# Autodesk Inventor assembly: X_CarriageR_V2_1
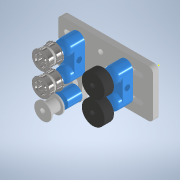
[picture p0: Inventor's stored thumbnail of the model, 180x180]
Saved by Autodesk Inventor 2021 (Build 250183000, 183)
## iProperties
Created: 2021-06-13
Part Number: X_CarriageR_V2_1
Document SubType Name: Assembly
Designer: Jorian Brusind
Author: Jorian Brusind
## Documents named in this file (9)
- C:\Users\Jorian Brusind\Documents\GitHub\PersonalProjects\HyperRail\Inventor Files\X_CarriageR_V2_1.iam
- C:\Users\Jorian Brusind\Documents\GitHub\PersonalProjects\HyperRail\Inventor Files\X_Carriage_Plate.ipt
- C:\Users\Jorian Brusind\Documents\GitHub\PersonalProjects\HyperRail\Inventor Files\Rollder_Spacer_Single.ipt
- C:\Users\Jorian Brusind\Documents\GitHub\PersonalProjects\HyperRail\Inventor Files\10mm_Idle_Pulley.ipt
- C:\Users\Jorian Brusind\Documents\GitHub\PersonalProjects\HyperRail\Inventor Files\4mm_Roller_Spacer_extended.ipt
- C:\Users\Jorian Brusind\Documents\GitHub\PersonalProjects\HyperRail\Inventor Files\11mm_BearingWheel.ipt
- C:\Users\Jorian Brusind\Documents\GitHub\PersonalProjects\HyperRail\Inventor Files\Bearing_Spacer.ipt
- C:\Users\Jorian Brusind\Documents\GitHub\PersonalProjects\HyperRail\Inventor Files\miniature-ball-bearings-metric-series-flanged-1.snapshot.1\F606ZZFlanged\F608 - 8 x 22 x 7.ipt
- C:\Users\Jorian Brusind\Documents\GitHub\PersonalProjects\HyperRail\Inventor Files\miniature-ball-bearings-metric-series-flanged-1.snapshot.1\F606ZZFlanged.ipt
## Components (13 placed, 7 different names)
1. X_Carriage_Plate:1 — Mate:35, Mate:67, Mate:69, Mate:72, Mate:84, Mate:85, Angle:1, Angle:2
2. Rollder_Spacer_Single:1 — Mate:35, Mate:40, Mate:42, Mate:67
3. 10mm_Idle_Pulley:1 — Mate:40, Mate:42
4. 4mm_Roller_Spacer_extended:1 — Mate:72, Mate:74, Mate:75, Mate:76, Mate:85, Angle:1
5. 4mm_Roller_Spacer_extended:3 — Mate:69, Mate:84, Angle:2, Mate:95, Mate:96, Mate:97
6. 11mm_BearingWheel:1 — Mate:75, Flush:1, Mate:76
7. 11mm_BearingWheel:2 — Mate:74, Flush:1
8. Bearing_Spacer:1 — Flush:3, Mate:92, Mate:93, Mate:94
9. Bearing_Spacer:2 — Flush:3, Mate:89, Mate:90, Mate:91
10. F608 - 8 x 22 x 7:1 — Mate:92, Mate:94, Mate:96
11. F608 - 8 x 22 x 7:2 — Mate:93
12. F608 - 8 x 22 x 7:3 — Mate:90
13. F608 - 8 x 22 x 7:4 — Mate:89, Mate:91, Mate:95, Mate:97
## Relationships (26: Mate 22, Flush 2, Angle 2)
- Mate:35: X_Carriage_Plate:1 ↔ Rollder_Spacer_Single:1
- Mate:40: Rollder_Spacer_Single:1 ↔ 10mm_Idle_Pulley:1
- Mate:42: Rollder_Spacer_Single:1 ↔ 10mm_Idle_Pulley:1
- Mate:67 (-18 mm): X_Carriage_Plate:1 ↔ Rollder_Spacer_Single:1
- Mate:69: X_Carriage_Plate:1 ↔ 4mm_Roller_Spacer_extended:3
- Mate:72: X_Carriage_Plate:1 ↔ 4mm_Roller_Spacer_extended:1
- Mate:74: 4mm_Roller_Spacer_extended:1 ↔ 11mm_BearingWheel:2
- Mate:75: 4mm_Roller_Spacer_extended:1 ↔ 11mm_BearingWheel:1
- Flush:1: 11mm_BearingWheel:1 ↔ 11mm_BearingWheel:2
- Mate:76: 4mm_Roller_Spacer_extended:1 ↔ 11mm_BearingWheel:1
- Mate:84 (-12.5 mm): X_Carriage_Plate:1 ↔ 4mm_Roller_Spacer_extended:3
- Mate:85 (-12.5 mm): X_Carriage_Plate:1 ↔ 4mm_Roller_Spacer_extended:1
- Angle:1 (0 deg): X_Carriage_Plate:1 ↔ 4mm_Roller_Spacer_extended:1
- Angle:2 (0 deg): X_Carriage_Plate:1 ↔ 4mm_Roller_Spacer_extended:3
- Flush:3: Bearing_Spacer:1 ↔ Bearing_Spacer:2
- [Mate]: F608 - 8 x 22 x 7:1 ↔ F608 - 8 x 22 x 7:2
- [Mate]: F608 - 8 x 22 x 7:3 ↔ F608 - 8 x 22 x 7:4
- Mate:89: Bearing_Spacer:2 ↔ F608 - 8 x 22 x 7:4
- Mate:90: Bearing_Spacer:2 ↔ F608 - 8 x 22 x 7:3
- Mate:91: Bearing_Spacer:2 ↔ F608 - 8 x 22 x 7:4
- Mate:92: Bearing_Spacer:1 ↔ F608 - 8 x 22 x 7:1
- Mate:93: Bearing_Spacer:1 ↔ F608 - 8 x 22 x 7:2
- Mate:94: Bearing_Spacer:1 ↔ F608 - 8 x 22 x 7:1
- Mate:95: 4mm_Roller_Spacer_extended:3 ↔ F608 - 8 x 22 x 7:4
- Mate:96: 4mm_Roller_Spacer_extended:3 ↔ F608 - 8 x 22 x 7:1
- Mate:97: 4mm_Roller_Spacer_extended:3 ↔ F608 - 8 x 22 x 7:4
## Named parameters: d136_d94 = 0 mm
